# Autodesk Inventor assembly: BatteryLatch
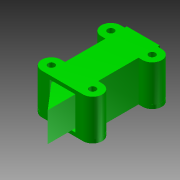
[picture p0: Inventor's stored thumbnail of the model, 180x180]
Saved by Autodesk Inventor 2012 (Build 160160000, 160)
## iProperties
Created: 2013-10-13
Part Number: BatteryLatch
Document SubType Name: Assembly
Designer: joe_000
Author: joe_000
## Documents named in this file (5)
- C:\dev\telepresenceRobot\mechanical\BatteryLatch.iam
- C:\dev\telepresenceRobot\mechanical\BatteryLatch-Outer.ipt
- C:\dev\telepresenceRobot\mechanical\BatteryLatch-Latch.ipt
- C:\dev\telepresenceRobot\mechanical\BatteryLatch-Spring.ipt
- C:\dev\telepresenceRobot\mechanical\BatteryLatch-Lower.ipt
## Components (4 placed, 4 different names)
1. BatteryLatch-Outer:1 — Insert:2, Angle:1, Mate:1, Insert:3, Insert:4
2. BatteryLatch-Latch:1 — Insert:1, Angle:1
3. BatteryLatch-Spring:1 — Insert:1, Insert:2
4. BatteryLatch-Lower:1 — Mate:1, Insert:3, Insert:4
## Relationships (6: Insert 4, Angle 1, Mate 1)
- Insert:1: BatteryLatch-Latch:1 ↔ BatteryLatch-Spring:1
- Insert:2: BatteryLatch-Outer:1 ↔ BatteryLatch-Spring:1
- Angle:1 (0 deg): BatteryLatch-Outer:1 ↔ BatteryLatch-Latch:1
- Mate:1: BatteryLatch-Outer:1 ↔ BatteryLatch-Lower:1
- Insert:3: BatteryLatch-Outer:1 ↔ BatteryLatch-Lower:1
- Insert:4: BatteryLatch-Outer:1 ↔ BatteryLatch-Lower:1
